# Autodesk Inventor assembly: Assembly3
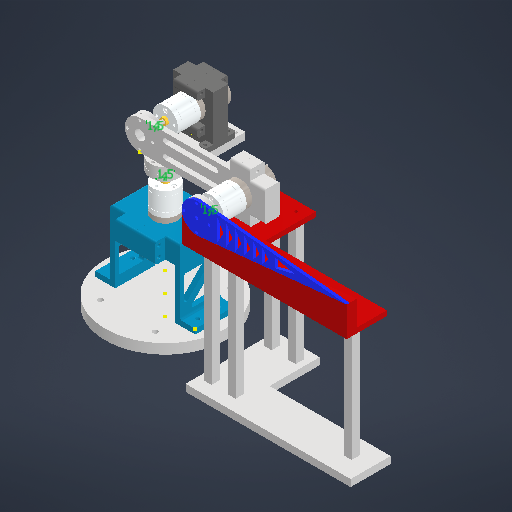
[picture p0: Inventor's stored thumbnail of the model, 512x512]
Saved by Autodesk Inventor 2026.1 (Build 301233020, 233B)
## iProperties
Created: 2026-04-08
Part Number: Assembly3
Document SubType Name: Assembly
Designer: kadir
Author: kadir
## Documents named in this file (14)
- C:\Users\kadir\Documents\erkin2\Assembly3.iam
- C:\Users\kadir\Documents\erkin2\alt gövde.ipt
- C:\Users\kadir\Documents\erkin2\motor dişlisi.ipt
- C:\Users\kadir\Desktop\25d-gearmotor-3d-models\25d-metal-gearmotor-75-99\25d-metal-gearmotor-75-99\25d-metal-gearmotor-75-99.ipt
- C:\Users\kadir\Documents\erkin2\alt blok.ipt
- C:\Users\kadir\Documents\erkin2\üst döner blok.ipt
- C:\Users\kadir\Documents\erkin2\üst döner tablo1.ipt
- C:\Users\kadir\Documents\erkin2\link1.ipt
- C:\Users\kadir\Documents\erkin2\motor kapak1.ipt
- C:\Users\kadir\Documents\erkin2\link2.ipt
- C:\Users\kadir\Documents\erkin2\TABAN base.ipt
- C:\Users\kadir\Documents\erkin2\2. parça\üst kısım.ipt
- C:\Users\kadir\Documents\erkin2\2. parça\bacaklar.ipt
- C:\Users\kadir\Documents\erkin2\2. parça\alt platform.ipt
## Components (23 placed, 13 different names)
1. alt gövde:1
2. 25d-metal-gearmotor-75-99:1 — Mate:4, Mate:6, Mate:7, Mate:8, Mate:51, Mate:52
3. 25d-metal-gearmotor-75-99:2 — Mate:30, Mate:31, Mate:32, Mate:33, Mate:34, Mate:35
4. 25d-metal-gearmotor-75-99:3 — Mate:42, Mate:43, Mate:44, Mate:45, Mate:46, Mate:47
5. alt blok:1 — Mate:4, Mate:52, Mate:53, Mate:54, Mate:55, Mate:57
6. alt blok:2 — Mate:51, Mate:53, Mate:54, Mate:55, Mate:56, Mate:58, Angle:4
7. motor dişlisi:1 — Mate:6, Mate:7, Mate:8, Mate:21, Mate:22, Mate:23
8. üst döner blok:1 — Mate:27, Mate:28, Mate:29, Mate:31, Angle:6
9. üst döner blok:2 — Mate:24, Mate:25, Mate:26, Mate:30, Mate:75
10. üst döner tablo1:1 — Mate:21, Mate:22, Mate:23, Mate:24, Mate:25, Mate:26, Mate:27, Mate:28, Mate:29, Angle:4, Mate:75
11. motor dişlisi:2 — Mate:32, Mate:33, Mate:34, Mate:36, Mate:37, Mate:38
12. link1:1 — Mate:35, Mate:36, Mate:37, Mate:38, Mate:39, Mate:40, Mate:41, Mate:42, Angle:1, Angle:2, Angle:6
13. motor kapak1:1 — Mate:39, Mate:40, Mate:41, Mate:43, Angle:5
14. motor dişlisi:3 — Mate:44, Mate:45, Mate:46, Mate:48, Mate:49, Mate:50
15. link2:1 — Mate:47, Mate:48, Mate:49, Mate:50, Angle:1, Angle:2, Angle:5, Mate:61, Mate:62
16. TABAN base:1 — Mate:56, Mate:57, Mate:58
17. üst kısım:1 — Mate:61, Mate:62, Mate:63, Mate:64, Mate:65, Mate:66, Mate:67, Mate:68, Mate:69, Mate:70, Mate:71, Mate:72, Angle:7, Angle:8, Angle:9, Angle:10, Angle:11
18. bacaklar:1 — Mate:66, Mate:72, Angle:8, Mate:74
19. bacaklar:2 — Mate:65, Mate:71, Angle:7
20. bacaklar:3 — Mate:64, Mate:69, Angle:10
21. bacaklar:4 — Mate:67, Mate:70, Angle:9, Mate:73
22. bacaklar:5 — Mate:63, Mate:68, Angle:11
23. alt platform:1 — Mate:73, Mate:74
## Relationships (67: Mate 57, Angle 10)
- Mate:4: 25d-metal-gearmotor-75-99:1 ↔ alt blok:1
- Mate:6: 25d-metal-gearmotor-75-99:1 ↔ motor dişlisi:1
- Mate:7: 25d-metal-gearmotor-75-99:1 ↔ motor dişlisi:1
- Mate:8: 25d-metal-gearmotor-75-99:1 ↔ motor dişlisi:1
- Mate:21: motor dişlisi:1 ↔ üst döner tablo1:1
- Mate:22: motor dişlisi:1 ↔ üst döner tablo1:1
- Mate:23: motor dişlisi:1 ↔ üst döner tablo1:1
- Mate:24: üst döner blok:2 ↔ üst döner tablo1:1
- Mate:25: üst döner blok:2 ↔ üst döner tablo1:1
- Mate:26: üst döner blok:2 ↔ üst döner tablo1:1
- Mate:27: üst döner blok:1 ↔ üst döner tablo1:1
- Mate:28: üst döner blok:1 ↔ üst döner tablo1:1
- Mate:29: üst döner blok:1 ↔ üst döner tablo1:1
- Mate:30: 25d-metal-gearmotor-75-99:2 ↔ üst döner blok:2
- Mate:31 (5 mm): 25d-metal-gearmotor-75-99:2 ↔ üst döner blok:1
- Mate:32: 25d-metal-gearmotor-75-99:2 ↔ motor dişlisi:2
- Mate:33: 25d-metal-gearmotor-75-99:2 ↔ motor dişlisi:2
- Mate:34 (3 mm): 25d-metal-gearmotor-75-99:2 ↔ motor dişlisi:2
- Mate:35: 25d-metal-gearmotor-75-99:2 ↔ link1:1
- Mate:36: motor dişlisi:2 ↔ link1:1
- Mate:37: motor dişlisi:2 ↔ link1:1
- Mate:38: motor dişlisi:2 ↔ link1:1
- Mate:39: link1:1 ↔ motor kapak1:1
- Mate:40: link1:1 ↔ motor kapak1:1
- Mate:41: link1:1 ↔ motor kapak1:1
- Mate:42: 25d-metal-gearmotor-75-99:3 ↔ link1:1
- Mate:43 (25 mm): 25d-metal-gearmotor-75-99:3 ↔ motor kapak1:1
- Mate:44: 25d-metal-gearmotor-75-99:3 ↔ motor dişlisi:3
- Mate:45: 25d-metal-gearmotor-75-99:3 ↔ motor dişlisi:3
- Mate:46 (2 mm): 25d-metal-gearmotor-75-99:3 ↔ motor dişlisi:3
- Mate:47: 25d-metal-gearmotor-75-99:3 ↔ link2:1
- Mate:48: motor dişlisi:3 ↔ link2:1
- Mate:49: motor dişlisi:3 ↔ link2:1
- Mate:50: motor dişlisi:3 ↔ link2:1
- Mate:51: 25d-metal-gearmotor-75-99:1 ↔ alt blok:2
- Mate:52 (25 mm): 25d-metal-gearmotor-75-99:1 ↔ alt blok:1
- Mate:53: alt blok:1 ↔ alt blok:2
- Mate:54: alt blok:1 ↔ alt blok:2
- Mate:55: alt blok:1 ↔ alt blok:2
- Mate:56: alt blok:2 ↔ TABAN base:1
- Mate:57: alt blok:1 ↔ TABAN base:1
- Mate:58: alt blok:2 ↔ TABAN base:1
- Angle:1 (0 deg): link1:1 ↔ link2:1
- Angle:2 (0 deg): link1:1 ↔ link2:1
- Angle:4 (0 deg): alt blok:2 ↔ üst döner tablo1:1
- Angle:5 (180 deg): motor kapak1:1 ↔ link2:1
- Angle:6 (180 deg): üst döner blok:1 ↔ link1:1
- Mate:61: link2:1 ↔ üst kısım:1
- Mate:62: link2:1 ↔ üst kısım:1
- Mate:63: üst kısım:1 ↔ bacaklar:5
- Mate:64: üst kısım:1 ↔ bacaklar:3
- Mate:65: üst kısım:1 ↔ bacaklar:2
- Mate:66: üst kısım:1 ↔ bacaklar:1
- Mate:67: üst kısım:1 ↔ bacaklar:4
- Mate:68: üst kısım:1 ↔ bacaklar:5
- Mate:69: üst kısım:1 ↔ bacaklar:3
- Mate:70: üst kısım:1 ↔ bacaklar:4
- Mate:71: üst kısım:1 ↔ bacaklar:2
- Mate:72: üst kısım:1 ↔ bacaklar:1
- Angle:7 (0 deg): üst kısım:1 ↔ bacaklar:2
- Angle:8 (0 deg): üst kısım:1 ↔ bacaklar:1
- Angle:9 (0 deg): üst kısım:1 ↔ bacaklar:4
- Angle:10 (0 deg): üst kısım:1 ↔ bacaklar:3
- Angle:11 (0 deg): üst kısım:1 ↔ bacaklar:5
- Mate:73: bacaklar:4 ↔ alt platform:1
- Mate:74: bacaklar:1 ↔ alt platform:1
- Mate:75: üst döner blok:2 ↔ üst döner tablo1:1
